# Autodesk Inventor assembly: Turntable New with Hole Base and Black Top
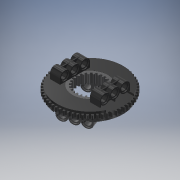
[picture p0: Inventor's stored thumbnail of the model, 180x180]
Saved by Autodesk Inventor 2018 (Build 220112000, 112)
## iProperties
Created: 2015-09-17
Part Number: Turntable New with Hole Base and Black Top
Document SubType Name: Assembly
Designer: herbi
Author: herbi
Sending System: SolidWorks 2012
Last Author: Martin
Last Saved: 2015-09-17
## Documents named in this file (3)
- D:\Lego 3D Files\lego-turntable-1.snapshot.1\Turntable New with Hole Base and Black Top.iam
- D:\Lego 3D Files\lego-turntable-1.snapshot.1\Top for Large Turntable.ipt
- D:\Lego 3D Files\lego-turntable-1.snapshot.1\Turntable Type 2 Base.ipt
## Components (2 placed, 2 different names)
1. Top for Large Turntable:1 — Insert:1
2. Turntable Type 2 Base:1 — Insert:1
## Relationships (1: Insert 1)
- Insert:1: Top for Large Turntable:1 ↔ Turntable Type 2 Base:1
